# Autodesk Inventor assembly: montagem-arcade4
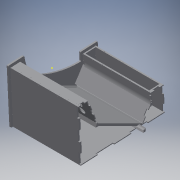
[picture p0: Inventor's stored thumbnail of the model, 180x180]
Saved by Autodesk Inventor 2016 (Build 200138000, 138)
## iProperties
Created: 2017-06-05
Part Number: montagem-arcade4
Material: Genérico
Document SubType Name: Assembly
Designer: Fabio
Author: Fabio
## Documents named in this file (15)
- C:\dev\arcade\montagem-arcade4.iam
- C:\dev\arcade\lateral.ipt
- C:\dev\arcade\traseira.ipt
- C:\dev\arcade\BASE.ipt
- C:\dev\arcade\frente inferior.ipt
- C:\dev\arcade\controles.ipt
- C:\dev\arcade\junta controler.ipt
- C:\dev\arcade\fechamento superior.ipt
- C:\dev\arcade\letreiro.ipt
- C:\dev\arcade\fechamento inferior.ipt
- C:\dev\arcade\junta auto falante.ipt
- C:\dev\arcade\placa auto falante.ipt
- C:\dev\arcade\tela.ipt
- C:\dev\arcade\juncao controle tela.ipt
- C:\dev\arcade\juncao tela - som.ipt
## Components (14 placed, 14 different names)
1. lateral:2 — Mate:3, Flush:5, Flush:6, Mate:9, Mate:12, Mate:15, Coincidência:21
2. traseira:1 — Mate:3, Flush:5, Flush:6, Mate:5, Flush:7, Mate:7, Mate:14, Flush:10, Alinhamento:22
3. BASE:1 — Mate:5, Flush:7, Mate:7, Mate:8, Flush:8, Coincidência:21
4. frente inferior:1 — Mate:8, Flush:8, Mate:9, Mate:10, Mate:11
5. junta controler:1 — Mate:10, Mate:11, Mate:12, Mate:13, Flush:9
6. controles:1 — Mate:13, Flush:9, Alinhamento:19
7. fechamento superior:1 — Mate:14, Flush:10, Mate:15, Flush:11, Flush:12, Mate:16, Alinhamento:21, Alinhamento:22
8. letreiro:1 — Flush:11, Flush:12, Mate:16, Flush:13, Mate:17, Flush:14, Alinhamento:21
9. fechamento inferior:1 — Flush:13, Mate:17, Flush:14, Alinhamento:16, Coincidência:19, Alinhamento:17
10. junta auto falante:1 — Coincidência:19, Alinhamento:17, Coincidência:20, Alinhamento:18
11. placa auto falante:1 — Alinhamento:16, Coincidência:20, Alinhamento:18
12. tela:1 — Alinhamento:20
13. juncao controle tela:1 — Alinhamento:19, Alinhamento:20
14. juncao tela - som:1
## Relationships (33: Flush 17, Mate 16)
- Mate:3 (-8 mm): lateral:2 ↔ traseira:1
- Flush:5: lateral:2 ↔ traseira:1
- Flush:6 (10 mm): lateral:2 ↔ traseira:1
- Mate:5 (-4 mm): traseira:1 ↔ BASE:1
- Flush:7: traseira:1 ↔ BASE:1
- Mate:7 (-4 mm): traseira:1 ↔ BASE:1
- Mate:8 (-8 mm): BASE:1 ↔ frente inferior:1
- Flush:8: BASE:1 ↔ frente inferior:1
- Mate:9 (-8 mm): lateral:2 ↔ frente inferior:1
- Mate:10: frente inferior:1 ↔ junta controler:1
- Mate:11: frente inferior:1 ↔ junta controler:1
- Mate:12: lateral:2 ↔ junta controler:1
- Mate:13: junta controler:1 ↔ controles:1
- Flush:9 (-8 mm): junta controler:1 ↔ controles:1
- Mate:14 (-4 mm): traseira:1 ↔ fechamento superior:1
- Flush:10: traseira:1 ↔ fechamento superior:1
- Mate:15 (-8 mm): lateral:2 ↔ fechamento superior:1
- Flush:11: fechamento superior:1 ↔ letreiro:1
- Flush:12: fechamento superior:1 ↔ letreiro:1
- Mate:16 (-4 mm): fechamento superior:1 ↔ letreiro:1
- Flush:13: letreiro:1 ↔ fechamento inferior:1
- Mate:17 (-4 mm): letreiro:1 ↔ fechamento inferior:1
- Flush:14: letreiro:1 ↔ fechamento inferior:1
- Alinhamento:16 [Flush]: fechamento inferior:1 ↔ placa auto falante:1
- Coincidência:19 [Mate]: fechamento inferior:1 ↔ junta auto falante:1
- Alinhamento:17 [Flush]: fechamento inferior:1 ↔ junta auto falante:1
- Coincidência:20 [Mate]: junta auto falante:1 ↔ placa auto falante:1
- Alinhamento:18 [Flush]: junta auto falante:1 ↔ placa auto falante:1
- Alinhamento:19 [Flush]: controles:1 ↔ juncao controle tela:1
- Alinhamento:20 [Flush]: tela:1 ↔ juncao controle tela:1
- Coincidência:21 [Mate] (-8 mm): lateral:2 ↔ BASE:1
- Alinhamento:21 [Flush]: fechamento superior:1 ↔ letreiro:1
- Alinhamento:22 [Flush]: traseira:1 ↔ fechamento superior:1
